# Autodesk Inventor assembly: Assembly1
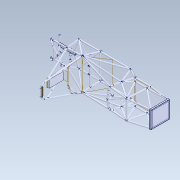
[picture p0: Inventor's stored thumbnail of the model, 180x180]
Saved by Autodesk Inventor 2021 (Build 250183000, 183)
## iProperties
Created: 2020-09-26
Part Number: Assembly1
Document SubType Name: Assembly
Designer: capta
Author: capta
## Documents named in this file (5)
- C:\Users\capta\OneDrive - Lehigh University\Formula SAE\Tractive Light\Assembly1.iam
- C:\Users\capta\OneDrive - Lehigh University\Formula SAE\Tractive Light\Mount CAD\LR-21-Chassis-1.0.0.ipt
- C:\Users\capta\OneDrive - Lehigh University\Formula SAE\Tractive Light\Mount CAD\Tractive Light Assembly.iam
- C:\Users\capta\OneDrive - Lehigh University\Formula SAE\Tractive Light\Tractive Light Enclosure 2.0.ipt
- C:\Users\capta\OneDrive - Lehigh University\Formula SAE\Tractive Light\Assembly2.iam
## Components (4 placed, 4 different names)
1. LR-21-Chassis-1.0.0:1 — Mate:1, Mate:2, Angle:2, Mate:3, Mate:4, Flush:2, Flush:3, Angle:3, Mate:5, Mate:7
2. Tractive Light Assembly:1 [sub-assembly] — Mate:1, Mate:2, Angle:1
3. Tractive Light Enclosure 2.0:1 — Flush:1, Mate:4
4. Assembly2:1 [sub-assembly] — Mate:6, Mate:7, Flush:4
## Relationships (14: Mate 7, Flush 4, Angle 3)
- Mate:1: LR-21-Chassis-1.0.0:1 ↔ Tractive Light Assembly:1
- Mate:2 (12.7 mm): LR-21-Chassis-1.0.0:1 ↔ Tractive Light Assembly:1
- Angle:1 (0 deg): Tractive Light Assembly:1
- Angle:2 (0 deg): LR-21-Chassis-1.0.0:1
- Mate:3: LR-21-Chassis-1.0.0:1
- Flush:1: Tractive Light Enclosure 2.0:1
- Mate:4: LR-21-Chassis-1.0.0:1 ↔ Tractive Light Enclosure 2.0:1
- Flush:2: LR-21-Chassis-1.0.0:1
- Flush:3 (-75 mm): LR-21-Chassis-1.0.0:1
- Angle:3 (0 deg): LR-21-Chassis-1.0.0:1
- Mate:5: LR-21-Chassis-1.0.0:1
- Mate:6: Assembly2:1
- Mate:7: LR-21-Chassis-1.0.0:1 ↔ Assembly2:1
- Flush:4: Assembly2:1
